# Autodesk Inventor assembly: robot
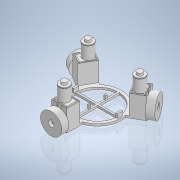
[picture p0: Inventor's stored thumbnail of the model, 180x180]
Saved by Autodesk Inventor 2020 (Build 240168000, 168)
## iProperties
Created: 2020-03-22
Part Number: robot
Document SubType Name: Assembly
Designer: Tarsoly
Author: Tarsoly
## Documents named in this file (4)
- D:\Users\Tarsoly\Dokumentumok\BME\8. Félév\Önlab\3d\robot.iam
- D:\Users\Tarsoly\Dokumentumok\BME\8. Félév\Önlab\3d\bottom.ipt
- D:\Users\Tarsoly\Dokumentumok\BME\8. Félév\Önlab\3d\motor.ipt
- D:\Users\Tarsoly\Dokumentumok\BME\8. Félév\Önlab\3d\omniwheel.ipt
## Components (7 placed, 3 different names)
1. bottom:1 — Mate:1, Mate:2, Angle:1, Mate:3, Mate:4, Mate:5, Angle:2, Mate:7, Mate:8, Mate:9, Angle:3, Mate:10, Mate:11
2. motor:1 — Mate:3, Mate:4, Flush:1, Mate:12
3. motor:2 — Flush:2, Mate:10, Mate:11, Mate:14
4. motor:3 — Mate:6, Mate:7, Mate:8, Mate:13
5. omniwheel:1 — Mate:12
6. omniwheel:2 — Mate:13
7. omniwheel:3 — Mate:14
## Relationships (19: Mate 14, Angle 3, Flush 2)
- Mate:1: bottom:1
- Mate:2: bottom:1
- Angle:1 (180 deg): bottom:1
- Mate:3: bottom:1 ↔ motor:1
- Mate:4: bottom:1 ↔ motor:1
- Flush:1 (16 mm): motor:1
- Mate:5: bottom:1
- Angle:2 (0 deg): bottom:1
- Mate:6 (-16 mm): motor:3
- Mate:7: bottom:1 ↔ motor:3
- Mate:8: bottom:1 ↔ motor:3
- Mate:9: bottom:1
- Angle:3 (0 deg): bottom:1
- Flush:2 (-16 mm): motor:2
- Mate:10: bottom:1 ↔ motor:2
- Mate:11: bottom:1 ↔ motor:2
- Mate:12: motor:1 ↔ omniwheel:1
- Mate:13: motor:3 ↔ omniwheel:2
- Mate:14: motor:2 ↔ omniwheel:3
